# Autodesk Inventor assembly: SinglePulley
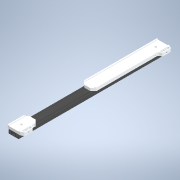
[picture p0: Inventor's stored thumbnail of the model, 180x180]
Saved by Autodesk Inventor 2020 (Build 240168000, 168)
## iProperties
Created: 2020-02-11
Part Number: SinglePulley
Document SubType Name: Assembly
Designer: maple
Author: maple
## Documents named in this file (4)
- C:\Users\maple\Documents\GitHub\CAD\Robotics 2019-2020\Assembly\PulleySystem\SinglePulley.iam
- C:\Users\maple\Documents\GitHub\CAD\Robotics 2019-2020\Assembly\PulleySystem\8x20x300mm-v2.ipt
- C:\Users\maple\Documents\GitHub\CAD\Robotics 2019-2020\Assembly\PulleySystem\3D-Print-Insert-Full-Multibody.ipt
- C:\Users\maple\Documents\GitHub\CAD\Robotics 2019-2020\Assembly\PulleySystem\3D-Print-Insert-Partial.ipt
## Components (3 placed, 3 different names)
1. 8x20x300mm-v2:1 — Rotational:1, Rotational:2, Flush:1, Flush:2, Flush:3, Flush:4
2. 3D-Print-Insert-Full-Multibody:1 — Rotational:1, Flush:2, Flush:3
3. 3D-Print-Insert-Partial:1 — Rotational:2, Flush:1, Flush:4
## Relationships (6: Flush 4, RevoluteJoint 2)
- Rotational:1 [RevoluteJoint]: 8x20x300mm-v2:1 ↔ 3D-Print-Insert-Full-Multibody:1
- Rotational:2 [RevoluteJoint]: 8x20x300mm-v2:1 ↔ 3D-Print-Insert-Partial:1
- Flush:1: 8x20x300mm-v2:1 ↔ 3D-Print-Insert-Partial:1
- Flush:2: 8x20x300mm-v2:1 ↔ 3D-Print-Insert-Full-Multibody:1
- Flush:3 (2.4892 mm): 8x20x300mm-v2:1 ↔ 3D-Print-Insert-Full-Multibody:1
- Flush:4 (2.4892 mm): 8x20x300mm-v2:1 ↔ 3D-Print-Insert-Partial:1
